# Autodesk Inventor assembly: 부피 구하기4
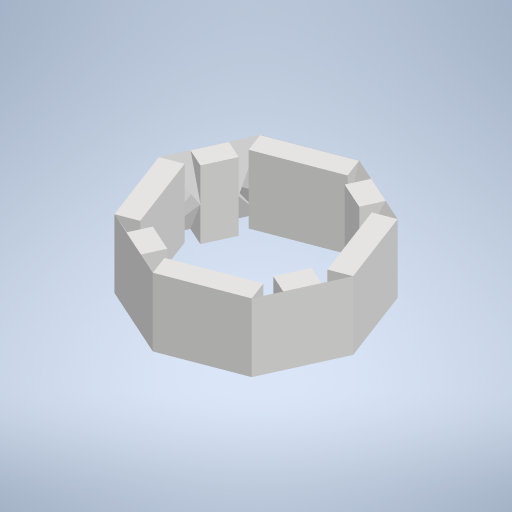
[picture p0: Inventor's stored thumbnail of the model, 512x512]
Saved by Autodesk Inventor 2024 (Build 280153000, 153)
## iProperties
Created: 2023-06-27
Part Number: 부피 구하기4
Document SubType Name: Assembly
Designer: jsw
Author: jsw
## Documents named in this file (4)
- C:\승원\co-op\OV-PAM\OV-PAM_modeling\부피 구하기4.iam
- C:\승원\co-op\OV-PAM\OV-PAM_modeling\부피 구하기2.ipt
- C:\승원\co-op\OV-PAM\OV-PAM_modeling\부피 구하기3.ipt
- C:\승원\co-op\OV-PAM\OV-PAM_modeling\부피 구하기6.ipt
## Components (9 placed, 3 different names)
1. 부피 구하기2:1 — 메이트:1, 메이트:3, 메이트:4, 메이트:6, 메이트:7, 메이트:9, 메이트:10, 메이트:12, 메이트:13, 메이트:15, 메이트:17, 메이트:19
2. 부피 구하기3:1 — 메이트:1, 메이트:3, 메이트:18
3. 부피 구하기3:2 — 메이트:10, 메이트:12, 메이트:14
4. 부피 구하기3:3 — 메이트:7, 메이트:9, 메이트:20
5. 부피 구하기3:4 — 메이트:4, 메이트:6, 메이트:16
6. 부피 구하기6:1 — 메이트:13, 메이트:14
7. 부피 구하기6:2 — 메이트:15, 메이트:16
8. 부피 구하기6:3 — 메이트:17, 메이트:18
9. 부피 구하기6:4 — 메이트:19, 메이트:20
## Relationships (16: Mate 16)
- 메이트:1 [Mate]: 부피 구하기2:1 ↔ 부피 구하기3:1
- 메이트:3 [Mate]: 부피 구하기2:1 ↔ 부피 구하기3:1
- 메이트:4 [Mate]: 부피 구하기2:1 ↔ 부피 구하기3:4
- 메이트:6 [Mate]: 부피 구하기2:1 ↔ 부피 구하기3:4
- 메이트:7 [Mate]: 부피 구하기2:1 ↔ 부피 구하기3:3
- 메이트:9 [Mate]: 부피 구하기2:1 ↔ 부피 구하기3:3
- 메이트:10 [Mate]: 부피 구하기2:1 ↔ 부피 구하기3:2
- 메이트:12 [Mate]: 부피 구하기2:1 ↔ 부피 구하기3:2
- 메이트:13 [Mate]: 부피 구하기2:1 ↔ 부피 구하기6:1
- 메이트:14 [Mate] (8.391 mm): 부피 구하기3:2 ↔ 부피 구하기6:1
- 메이트:15 [Mate]: 부피 구하기2:1 ↔ 부피 구하기6:2
- 메이트:16 [Mate] (8.391 mm): 부피 구하기3:4 ↔ 부피 구하기6:2
- 메이트:17 [Mate]: 부피 구하기2:1 ↔ 부피 구하기6:3
- 메이트:18 [Mate] (8.391 mm): 부피 구하기3:1 ↔ 부피 구하기6:3
- 메이트:19 [Mate]: 부피 구하기2:1 ↔ 부피 구하기6:4
- 메이트:20 [Mate] (8.391 mm): 부피 구하기3:3 ↔ 부피 구하기6:4
